# Autodesk Inventor assembly: chassis
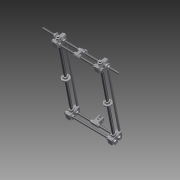
[picture p0: Inventor's stored thumbnail of the model, 180x180]
Saved by Autodesk Inventor 2015 (Build 190159000, 159)
## iProperties
Created: 2015-04-28
Part Number: chassis
Document SubType Name: Assembly
Designer: X
Author: X
## Documents named in this file (9)
- G:\3d printer\Prusa i3\CAD\chassis.iam
- G:\3d printer\Prusa i3\CAD\Y-idler.iam
- G:\3d printer\Prusa i3\CAD\rod\M8-205.ipt
- D:\Inventor\Content Center Files\R2015\en-US\ISO 7089\ISO 7089 - 8 - 140 HV(1).ipt
- D:\Inventor\Content Center Files\R2015\en-US\DIN 934\DIN 934 - M8 x 1.25.ipt
- G:\3d printer\Prusa i3\CAD\port_starboard_side.iam
- G:\3d printer\Prusa i3\CAD\3d_printer_part\y-motor.ipt
- G:\3d printer\Prusa i3\CAD\rod\M8-310.ipt
- D:\Inventor\Content Center Files\R2015\en-US\ISO 7093 A\ISO 7093 A - ST 8 - 140 HV .ipt
## Components (58 placed, 8 different names)
1. Y-idler:1 [sub-assembly] — Cylindrical:1, Insert:1, Insert:2, Angle:1
2. M8-205:1 — Cylindrical:1, Cylindrical:2, Cylindrical:3, Cylindrical:4, Cylindrical:5, Cylindrical:16, Cylindrical:18, Cylindrical:20, Cylindrical:21
3. ISO 7089 8 - 140 HV:1 — Insert:1, Mate:1
4. ISO 7089 8 - 140 HV:2 — Insert:2, Mate:2
5. DIN 934 - replaced by DIN EN 24032/28673/28674 M8:1 — Cylindrical:2, Mate:1
6. DIN 934 - replaced by DIN EN 24032/28673/28674 M8:2 — Cylindrical:3, Mate:2
7. port_starboard_side:1 [sub-assembly] — Cylindrical:4, Cylindrical:7, Mate:7, Mate:8, Mate:9, Mate:10, Cylindrical:27, Mate:19, Mate:20, Mate:21, Mate:22, Angle:1
8. port_starboard_side:2 [sub-assembly] — Cylindrical:5, Cylindrical:6, Mate:6, Mate:23, Mate:24, Mate:25, Mate:26
9. M8-205:2 — Cylindrical:6, Cylindrical:7, Cylindrical:17, Cylindrical:19, Cylindrical:22, Cylindrical:23
10. ISO 7089 8 - 140 HV:3 — Mate:6, Mate:12
11. ISO 7089 8 - 140 HV:4 — Mate:7, Mate:16
12. ISO 7089 8 - 140 HV:5 — Mate:11
13. ISO 7089 8 - 140 HV:6 — Mate:9, Mate:17
14. ISO 7089 8 - 140 HV:7 — Mate:10, Mate:18
15. ISO 7089 8 - 140 HV:8 — Mate:8, Mate:15
16. ISO 7089 8 - 140 HV:9 — Mate:13
17. ISO 7089 8 - 140 HV:10 — Mate:14
18. DIN 934 - replaced by DIN EN 24032/28673/28674 M8:3 — Cylindrical:16, Mate:17
19. DIN 934 - replaced by DIN EN 24032/28673/28674 M8:4 — Cylindrical:18, Mate:16
20. DIN 934 - replaced by DIN EN 24032/28673/28674 M8:5 — Cylindrical:17, Mate:18
21. DIN 934 - replaced by DIN EN 24032/28673/28674 M8:6 — Cylindrical:19, Mate:12
22. DIN 934 - replaced by DIN EN 24032/28673/28674 M8:7 — Cylindrical:21, Mate:11
23. DIN 934 - replaced by DIN EN 24032/28673/28674 M8:8 — Cylindrical:23, Mate:15
24. DIN 934 - replaced by DIN EN 24032/28673/28674 M8:9 — Cylindrical:20, Mate:13
25. DIN 934 - replaced by DIN EN 24032/28673/28674 M8:10 — Cylindrical:22, Mate:14
26. y-motor:1 — Cylindrical:25, Mate:27, Mate:28, Mate:29, Mate:30
27. M8-310:1 — Cylindrical:52, Cylindrical:53, Cylindrical:54, Cylindrical:55, Cylindrical:56, Cylindrical:57
28. M8-205:3 — Cylindrical:25, Cylindrical:27, Cylindrical:29, Cylindrical:31, Cylindrical:33, Cylindrical:35, Cylindrical:36, Cylindrical:39, Cylindrical:41, Cylindrical:44, Cylindrical:45, Cylindrical:48, Cylindrical:49, Cylindrical:51
29. ISO 7089 8 - 140 HV:11 — Mate:26, Mate:31
30. ISO 7089 8 - 140 HV:12 — Cylindrical:29, Mate:25, Mate:32
31. ISO 7089 8 - 140 HV:13 — Mate:23, Mate:34
32. ISO 7089 8 - 140 HV:14 — Cylindrical:31, Mate:24, Mate:33
33. ISO 7089 8 - 140 HV:15 — Mate:19, Mate:42
34. ISO 7089 8 - 140 HV:16 — Mate:21, Mate:39
35. ISO 7089 8 - 140 HV:17 — Cylindrical:35, Mate:20, Mate:41
36. ISO 7089 8 - 140 HV:18 — Cylindrical:33, Mate:22, Mate:40
37. ISO 7089 8 - 140 HV:19 — Cylindrical:36, Mate:30, Mate:38
38. ISO 7089 8 - 140 HV:20 — Cylindrical:39, Mate:29, Mate:35
39. ISO 7089 8 - 140 HV:21 — Mate:27, Mate:36
40. ISO 7089 8 - 140 HV:22 — Mate:28, Mate:37
41. DIN 934 - replaced by DIN EN 24032/28673/28674 M8:11 — Mate:31, Mate:45
42. DIN 934 - replaced by DIN EN 24032/28673/28674 M8:12 — Cylindrical:41, Mate:32
43. DIN 934 - replaced by DIN EN 24032/28673/28674 M8:13 — Mate:36
44. DIN 934 - replaced by DIN EN 24032/28673/28674 M8:14 — Mate:34
45. DIN 934 - replaced by DIN EN 24032/28673/28674 M8:15 — Cylindrical:45, Mate:33
46. DIN 934 - replaced by DIN EN 24032/28673/28674 M8:16 — Cylindrical:44, Mate:35
47. DIN 934 - replaced by DIN EN 24032/28673/28674 M8:17 — Mate:37
48. DIN 934 - replaced by DIN EN 24032/28673/28674 M8:18 — Cylindrical:48, Mate:40
49. DIN 934 - replaced by DIN EN 24032/28673/28674 M8:19 — Mate:42, Mate:43
50. DIN 934 - replaced by DIN EN 24032/28673/28674 M8:20 — Cylindrical:49, Mate:38
51. DIN 934 - replaced by DIN EN 24032/28673/28674 M8:21 — Mate:39
52. DIN 934 - replaced by DIN EN 24032/28673/28674 M8:22 — Cylindrical:51, Mate:41
53. ISO 7093 A ST 8 - 140 HV - A:1 — Cylindrical:52, Mate:44, Mate:48
54. ISO 7093 A ST 8 - 140 HV - A:2 — Cylindrical:53, Mate:43, Mate:44
55. ISO 7093 A ST 8 - 140 HV - A:3 — Cylindrical:54, Mate:45, Mate:46
56. ISO 7093 A ST 8 - 140 HV - A:4 — Cylindrical:55, Mate:46, Mate:47
57. DIN 934 - replaced by DIN EN 24032/28673/28674 M8:23 — Cylindrical:56, Mate:48
58. DIN 934 - replaced by DIN EN 24032/28673/28674 M8:24 — Cylindrical:57, Mate:47
## Relationships (108: CylindricalJoint 57, Mate 48, Insert 2, Angle 1)
- Cylindrical:1: Y-idler:1 ↔ M8-205:1
- Insert:1: Y-idler:1 ↔ ISO 7089 8 - 140 HV:1
- Insert:2: Y-idler:1 ↔ ISO 7089 8 - 140 HV:2
- Cylindrical:2: M8-205:1 ↔ DIN 934 - replaced by DIN EN 24032/28673/28674 M8:1
- Mate:1: ISO 7089 8 - 140 HV:1 ↔ DIN 934 - replaced by DIN EN 24032/28673/28674 M8:1
- Cylindrical:3: M8-205:1 ↔ DIN 934 - replaced by DIN EN 24032/28673/28674 M8:2
- Mate:2: ISO 7089 8 - 140 HV:2 ↔ DIN 934 - replaced by DIN EN 24032/28673/28674 M8:2
- Cylindrical:4: M8-205:1 ↔ port_starboard_side:1
- Cylindrical:5: M8-205:1 ↔ port_starboard_side:2
- Cylindrical:6: port_starboard_side:2 ↔ M8-205:2
- Cylindrical:7: port_starboard_side:1 ↔ M8-205:2
- [CylindricalJoint]: M8-205:1 ↔ ISO 7089 8 - 140 HV:5
- [CylindricalJoint]: M8-205:1 ↔ ISO 7089 8 - 140 HV:4
- [CylindricalJoint]: M8-205:1 ↔ ISO 7089 8 - 140 HV:6
- [CylindricalJoint]: M8-205:2 ↔ ISO 7089 8 - 140 HV:3
- [CylindricalJoint]: M8-205:2 ↔ ISO 7089 8 - 140 HV:8
- [CylindricalJoint]: M8-205:2 ↔ ISO 7089 8 - 140 HV:7
- [CylindricalJoint]: M8-205:1 ↔ ISO 7089 8 - 140 HV:9
- [CylindricalJoint]: M8-205:2 ↔ ISO 7089 8 - 140 HV:10
- [Mate]: port_starboard_side:2 ↔ ISO 7089 8 - 140 HV:9
- [Mate]: port_starboard_side:2 ↔ ISO 7089 8 - 140 HV:10
- [Mate]: port_starboard_side:2 ↔ ISO 7089 8 - 140 HV:5
- Mate:6: port_starboard_side:2 ↔ ISO 7089 8 - 140 HV:3
- Mate:7: port_starboard_side:1 ↔ ISO 7089 8 - 140 HV:4
- Mate:8: port_starboard_side:1 ↔ ISO 7089 8 - 140 HV:8
- Mate:9: port_starboard_side:1 ↔ ISO 7089 8 - 140 HV:6
- Mate:10: port_starboard_side:1 ↔ ISO 7089 8 - 140 HV:7
- Cylindrical:16: M8-205:1 ↔ DIN 934 - replaced by DIN EN 24032/28673/28674 M8:3
- Cylindrical:17: M8-205:2 ↔ DIN 934 - replaced by DIN EN 24032/28673/28674 M8:5
- Cylindrical:18: M8-205:1 ↔ DIN 934 - replaced by DIN EN 24032/28673/28674 M8:4
- Cylindrical:19: M8-205:2 ↔ DIN 934 - replaced by DIN EN 24032/28673/28674 M8:6
- Cylindrical:20: M8-205:1 ↔ DIN 934 - replaced by DIN EN 24032/28673/28674 M8:9
- Cylindrical:21: M8-205:1 ↔ DIN 934 - replaced by DIN EN 24032/28673/28674 M8:7
- Cylindrical:22: M8-205:2 ↔ DIN 934 - replaced by DIN EN 24032/28673/28674 M8:10
- Cylindrical:23: M8-205:2 ↔ DIN 934 - replaced by DIN EN 24032/28673/28674 M8:8
- Mate:11: ISO 7089 8 - 140 HV:5 ↔ DIN 934 - replaced by DIN EN 24032/28673/28674 M8:7
- Mate:12: ISO 7089 8 - 140 HV:3 ↔ DIN 934 - replaced by DIN EN 24032/28673/28674 M8:6
- Mate:13: ISO 7089 8 - 140 HV:9 ↔ DIN 934 - replaced by DIN EN 24032/28673/28674 M8:9
- Mate:14: ISO 7089 8 - 140 HV:10 ↔ DIN 934 - replaced by DIN EN 24032/28673/28674 M8:10
- Mate:15: ISO 7089 8 - 140 HV:8 ↔ DIN 934 - replaced by DIN EN 24032/28673/28674 M8:8
- Mate:16: ISO 7089 8 - 140 HV:4 ↔ DIN 934 - replaced by DIN EN 24032/28673/28674 M8:4
- Mate:17: ISO 7089 8 - 140 HV:6 ↔ DIN 934 - replaced by DIN EN 24032/28673/28674 M8:3
- Mate:18: ISO 7089 8 - 140 HV:7 ↔ DIN 934 - replaced by DIN EN 24032/28673/28674 M8:5
- [CylindricalJoint]: y-motor:1 ↔ M8-310:1
- Cylindrical:25: y-motor:1 ↔ M8-205:3
- [CylindricalJoint]: port_starboard_side:2 ↔ M8-310:1
- Cylindrical:27: port_starboard_side:1 ↔ M8-205:3
- [CylindricalJoint]: M8-310:1 ↔ ISO 7089 8 - 140 HV:11
- Cylindrical:29: M8-205:3 ↔ ISO 7089 8 - 140 HV:12
- [CylindricalJoint]: M8-310:1 ↔ ISO 7089 8 - 140 HV:13
- Cylindrical:31: M8-205:3 ↔ ISO 7089 8 - 140 HV:14
- [CylindricalJoint]: M8-310:1 ↔ ISO 7089 8 - 140 HV:16
- Cylindrical:33: M8-205:3 ↔ ISO 7089 8 - 140 HV:18
- [CylindricalJoint]: M8-310:1 ↔ ISO 7089 8 - 140 HV:15
- Cylindrical:35: M8-205:3 ↔ ISO 7089 8 - 140 HV:17
- Mate:19: port_starboard_side:1 ↔ ISO 7089 8 - 140 HV:15
- Mate:20: port_starboard_side:1 ↔ ISO 7089 8 - 140 HV:17
- Mate:21: port_starboard_side:1 ↔ ISO 7089 8 - 140 HV:16
- Mate:22: port_starboard_side:1 ↔ ISO 7089 8 - 140 HV:18
- Mate:23: port_starboard_side:2 ↔ ISO 7089 8 - 140 HV:13
- Mate:24: port_starboard_side:2 ↔ ISO 7089 8 - 140 HV:14
- Mate:25: port_starboard_side:2 ↔ ISO 7089 8 - 140 HV:12
- Mate:26: port_starboard_side:2 ↔ ISO 7089 8 - 140 HV:11
- Cylindrical:36: M8-205:3 ↔ ISO 7089 8 - 140 HV:19
- [CylindricalJoint]: M8-310:1 ↔ ISO 7089 8 - 140 HV:21
- [CylindricalJoint]: M8-310:1 ↔ ISO 7089 8 - 140 HV:22
- Cylindrical:39: M8-205:3 ↔ ISO 7089 8 - 140 HV:20
- Mate:27: y-motor:1 ↔ ISO 7089 8 - 140 HV:21
- Mate:28: y-motor:1 ↔ ISO 7089 8 - 140 HV:22
- Mate:29: y-motor:1 ↔ ISO 7089 8 - 140 HV:20
- Mate:30: y-motor:1 ↔ ISO 7089 8 - 140 HV:19
- [CylindricalJoint]: M8-310:1 ↔ DIN 934 - replaced by DIN EN 24032/28673/28674 M8:11
- Cylindrical:41: M8-205:3 ↔ DIN 934 - replaced by DIN EN 24032/28673/28674 M8:12
- [CylindricalJoint]: M8-310:1 ↔ DIN 934 - replaced by DIN EN 24032/28673/28674 M8:14
- [CylindricalJoint]: M8-310:1 ↔ DIN 934 - replaced by DIN EN 24032/28673/28674 M8:13
- Cylindrical:44: M8-205:3 ↔ DIN 934 - replaced by DIN EN 24032/28673/28674 M8:16
- Cylindrical:45: M8-205:3 ↔ DIN 934 - replaced by DIN EN 24032/28673/28674 M8:15
- [CylindricalJoint]: M8-310:1 ↔ DIN 934 - replaced by DIN EN 24032/28673/28674 M8:19
- [CylindricalJoint]: M8-310:1 ↔ DIN 934 - replaced by DIN EN 24032/28673/28674 M8:17
- Cylindrical:48: M8-205:3 ↔ DIN 934 - replaced by DIN EN 24032/28673/28674 M8:18
- Cylindrical:49: M8-205:3 ↔ DIN 934 - replaced by DIN EN 24032/28673/28674 M8:20
- [CylindricalJoint]: M8-310:1 ↔ DIN 934 - replaced by DIN EN 24032/28673/28674 M8:21
- Cylindrical:51: M8-205:3 ↔ DIN 934 - replaced by DIN EN 24032/28673/28674 M8:22
- Mate:31: ISO 7089 8 - 140 HV:11 ↔ DIN 934 - replaced by DIN EN 24032/28673/28674 M8:11
- Mate:32: ISO 7089 8 - 140 HV:12 ↔ DIN 934 - replaced by DIN EN 24032/28673/28674 M8:12
- Mate:33: ISO 7089 8 - 140 HV:14 ↔ DIN 934 - replaced by DIN EN 24032/28673/28674 M8:15
- Mate:34: ISO 7089 8 - 140 HV:13 ↔ DIN 934 - replaced by DIN EN 24032/28673/28674 M8:14
- Mate:35: ISO 7089 8 - 140 HV:20 ↔ DIN 934 - replaced by DIN EN 24032/28673/28674 M8:16
- Mate:36: ISO 7089 8 - 140 HV:21 ↔ DIN 934 - replaced by DIN EN 24032/28673/28674 M8:13
- Mate:37: ISO 7089 8 - 140 HV:22 ↔ DIN 934 - replaced by DIN EN 24032/28673/28674 M8:17
- Mate:38: ISO 7089 8 - 140 HV:19 ↔ DIN 934 - replaced by DIN EN 24032/28673/28674 M8:20
- Mate:39: ISO 7089 8 - 140 HV:16 ↔ DIN 934 - replaced by DIN EN 24032/28673/28674 M8:21
- Mate:40: ISO 7089 8 - 140 HV:18 ↔ DIN 934 - replaced by DIN EN 24032/28673/28674 M8:18
- Mate:41: ISO 7089 8 - 140 HV:17 ↔ DIN 934 - replaced by DIN EN 24032/28673/28674 M8:22
- Mate:42: ISO 7089 8 - 140 HV:15 ↔ DIN 934 - replaced by DIN EN 24032/28673/28674 M8:19
- Angle:1 (0 deg): Y-idler:1 ↔ port_starboard_side:1
- Cylindrical:52: M8-310:1 ↔ ISO 7093 A ST 8 - 140 HV - A:1
- Cylindrical:53: M8-310:1 ↔ ISO 7093 A ST 8 - 140 HV - A:2
- Cylindrical:54: M8-310:1 ↔ ISO 7093 A ST 8 - 140 HV - A:3
- Cylindrical:55: M8-310:1 ↔ ISO 7093 A ST 8 - 140 HV - A:4
- Mate:43: DIN 934 - replaced by DIN EN 24032/28673/28674 M8:19 ↔ ISO 7093 A ST 8 - 140 HV - A:2
- Mate:44: ISO 7093 A ST 8 - 140 HV - A:1 ↔ ISO 7093 A ST 8 - 140 HV - A:2
- Mate:45: DIN 934 - replaced by DIN EN 24032/28673/28674 M8:11 ↔ ISO 7093 A ST 8 - 140 HV - A:3
- Mate:46: ISO 7093 A ST 8 - 140 HV - A:3 ↔ ISO 7093 A ST 8 - 140 HV - A:4
- Cylindrical:56: M8-310:1 ↔ DIN 934 - replaced by DIN EN 24032/28673/28674 M8:23
- Cylindrical:57: M8-310:1 ↔ DIN 934 - replaced by DIN EN 24032/28673/28674 M8:24
- Mate:47: ISO 7093 A ST 8 - 140 HV - A:4 ↔ DIN 934 - replaced by DIN EN 24032/28673/28674 M8:24
- Mate:48: ISO 7093 A ST 8 - 140 HV - A:1 ↔ DIN 934 - replaced by DIN EN 24032/28673/28674 M8:23
